# Autodesk Inventor assembly: Plate 1
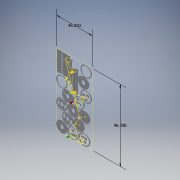
[picture p0: Inventor's stored thumbnail of the model, 180x180]
Saved by Autodesk Inventor 2016 (Build 200138000, 138)
## iProperties
Created: 2016-04-26
Part Number: Plate 1
Document SubType Name: Assembly
Designer: rubenjm
Author: rubenjm
## Documents named in this file (14)
- C:\Users\rubenjm\Documents\To Transfer\2k16 Spring\RME\GGC\V3\Plate 1.iam
- C:\Users\rubenjm\Documents\To Transfer\2k16 Spring\RME\GGC\V3\Arm Base.ipt
- C:\Users\rubenjm\Documents\To Transfer\2k16 Spring\RME\GGC\V3\Holder.ipt
- C:\Users\rubenjm\Documents\To Transfer\2k16 Spring\RME\GGC\V3\Far End Cap.ipt
- C:\Users\rubenjm\Documents\To Transfer\2k16 Spring\RME\GGC\V3\Near Holder.ipt
- C:\Users\rubenjm\Documents\To Transfer\2k16 Spring\RME\GGC\V3\Motor Bracket.ipt
- C:\Users\rubenjm\Documents\To Transfer\2k16 Spring\RME\GGC\V3\Near End Cap.ipt
- C:\Users\rubenjm\Documents\To Transfer\2k16 Spring\RME\GGC\V3\Arm Side.ipt
- C:\Users\rubenjm\Documents\To Transfer\2k16 Spring\RME\GGC\V3\Arm Top.ipt
- C:\Users\rubenjm\Documents\To Transfer\2k16 Spring\RME\GGC\V3\Turntable Top.ipt
- C:\Users\rubenjm\Documents\To Transfer\2k16 Spring\RME\GGC\V3\Turntable Sheath.ipt
- C:\Users\rubenjm\Documents\To Transfer\2k16 Spring\RME\GGC\V3\Turntable Mount.ipt
- C:\Users\rubenjm\Documents\To Transfer\2k16 Spring\RME\GGC\V3\Turntable Cap.ipt
- C:\Users\rubenjm\Documents\To Transfer\2k16 Spring\RME\GGC\V3\Turntable Mid.ipt
## Components (36 placed, 13 different names)
1. Arm Base:1 — Mate:1, Mate:59, Mate:75, Tangent:36
2. Holder:1 — Mate:4
3. Holder:2 — Mate:7
4. Far End Cap:1 — Mate:10
5. Near Holder:1 — Mate:13
6. Motor Bracket:1 — Mate:17
7. Near End Cap:1 — Mate:21
8. Arm Side:1 — Mate:25, Mate:64, Mate:69, Mate:70
9. Arm Side:2 — Mate:28, Mate:61, Mate:66, Mate:70, Mate:71
10. Arm Top:1 — Mate:30, Mate:60, Mate:72, Mate:73
11. Turntable Top:1 — Mate:33, Tangent:1, Tangent:2, Tangent:4, Tangent:10
12. Turntable Sheath:1 — Mate:34, Tangent:9, Tangent:10, Mate:41, Tangent:13, Tangent:34
13. Turntable Sheath:2 — Mate:38, Tangent:3, Tangent:4, Tangent:6, Tangent:9
14. Turntable Sheath:3 — Mate:37, Tangent:5, Tangent:6, Tangent:35
15. Turntable Sheath:4 — Mate:36, Tangent:32
16. Turntable Mount:1 — Mate:35, Mate:41
17. Turntable Cap:1 — Mate:40, Tangent:16, Tangent:19, Tangent:26
18. Turntable Mid:1 — Mate:39, Tangent:31, Tangent:32, Tangent:36
19. Arm Base:2 — Mate:55, Mate:74, Mate:75
20. Holder:3 — Mate:63
21. Holder:4 — Mate:57
22. Far End Cap:2 — Mate:53
23. Near Holder:2 — Mate:62
24. Motor Bracket:2 — Mate:52
25. Near End Cap:2 — Mate:54
26. Arm Side:3 — Mate:58, Mate:68, Mate:69
27. Arm Side:4 — Mate:65, Mate:71, Mate:72
28. Arm Top:2 — Mate:56, Mate:73, Mate:74
29. Turntable Top:2 — Tangent:13, Tangent:16, Tangent:18, Tangent:20, Mate:45, Tangent:33
30. Turntable Sheath:5 — Mate:44, Tangent:29, Tangent:30
31. Turntable Sheath:6 — Mate:43, Tangent:21, Tangent:22, Mate:50, Mate:67, Mate:76, Tangent:34
32. Turntable Sheath:7 — Mate:48, Tangent:26, Tangent:27, Tangent:28, Tangent:33
33. Turntable Sheath:8 — Mate:51, Tangent:28, Tangent:31
34. Turntable Mount:2 — Mate:46, Mate:76
35. Turntable Cap:2 — Mate:42, Tangent:19, Tangent:20, Tangent:35
36. Turntable Mid:2 — Tangent:18, Tangent:22, Mate:49, Tangent:27, Tangent:30
## Relationships (79: Mate 53, Tangent 26)
- Mate:1: Arm Base:1
- Mate:4: Holder:1
- Mate:7: Holder:2
- Mate:10: Far End Cap:1
- Mate:13: Near Holder:1
- Mate:17: Motor Bracket:1
- Mate:21: Near End Cap:1
- Mate:25: Arm Side:1
- Mate:28: Arm Side:2
- Mate:30: Arm Top:1
- Mate:33: Turntable Top:1
- Mate:34: Turntable Sheath:1
- Mate:35: Turntable Mount:1
- Mate:36: Turntable Sheath:4
- Mate:37: Turntable Sheath:3
- Mate:38: Turntable Sheath:2
- Mate:39: Turntable Mid:1
- Mate:40: Turntable Cap:1
- Tangent:1: Turntable Top:1
- Tangent:2: Turntable Top:1
- Tangent:3: Turntable Sheath:2
- Tangent:4 (6.35 mm): Turntable Top:1 ↔ Turntable Sheath:2
- Tangent:5: Turntable Sheath:3
- Tangent:6 (6.35 mm): Turntable Sheath:2 ↔ Turntable Sheath:3
- Tangent:9 (6.35 mm): Turntable Sheath:1 ↔ Turntable Sheath:2
- Tangent:10 (6.35 mm): Turntable Top:1 ↔ Turntable Sheath:1
- Mate:41: Turntable Sheath:1 ↔ Turntable Mount:1
- Tangent:13 (6.35 mm): Turntable Sheath:1 ↔ Turntable Top:2
- Tangent:16 (6.35 mm): Turntable Cap:1 ↔ Turntable Top:2
- Tangent:18 (6.35 mm): Turntable Top:2 ↔ Turntable Mid:2
- Mate:42: Turntable Cap:2
- Tangent:19 (6.35 mm): Turntable Cap:1 ↔ Turntable Cap:2
- Tangent:20 (6.35 mm): Turntable Top:2 ↔ Turntable Cap:2
- Mate:43: Turntable Sheath:6
- Tangent:21: Turntable Sheath:6
- Tangent:22 (6.35 mm): Turntable Sheath:6 ↔ Turntable Mid:2
- Mate:44: Turntable Sheath:5
- Mate:45: Turntable Top:2
- Mate:46: Turntable Mount:2
- Mate:48: Turntable Sheath:7
- Mate:49: Turntable Mid:2
- Tangent:26 (6.35 mm): Turntable Cap:1 ↔ Turntable Sheath:7
- Tangent:27 (6.35 mm): Turntable Sheath:7 ↔ Turntable Mid:2
- Mate:50: Turntable Sheath:6
- Mate:51: Turntable Sheath:8
- Tangent:28 (6.35 mm): Turntable Sheath:7 ↔ Turntable Sheath:8
- Mate:52: Motor Bracket:2
- Mate:53: Far End Cap:2
- Mate:54: Near End Cap:2
- Mate:55: Arm Base:2
- Mate:56: Arm Top:2
- Mate:57: Holder:4
- Mate:58: Arm Side:3
- Mate:59: Arm Base:1
- Mate:60: Arm Top:1
- Mate:61: Arm Side:2
- Mate:62: Near Holder:2
- Mate:63: Holder:3
- Mate:64: Arm Side:1
- Mate:65: Arm Side:4
- Mate:66: Arm Side:2
- Mate:67: Turntable Sheath:6
- Tangent:29: Turntable Sheath:5
- Tangent:30 (6.35 mm): Turntable Sheath:5 ↔ Turntable Mid:2
- Tangent:31 (6.35 mm): Turntable Mid:1 ↔ Turntable Sheath:8
- Mate:68: Arm Side:3
- Mate:69 (6.35 mm): Arm Side:1 ↔ Arm Side:3
- Mate:70 (6.35 mm): Arm Side:1 ↔ Arm Side:2
- Mate:71 (6.35 mm): Arm Side:2 ↔ Arm Side:4
- Mate:72 (6.35 mm): Arm Top:1 ↔ Arm Side:4
- Mate:73 (6.35 mm): Arm Top:1 ↔ Arm Top:2
- Mate:74 (6.35 mm): Arm Base:2 ↔ Arm Top:2
- Mate:75 (6.35 mm): Arm Base:1 ↔ Arm Base:2
- Tangent:32 (6.35 mm): Turntable Sheath:4 ↔ Turntable Mid:1
- Tangent:33 (6.35 mm): Turntable Top:2 ↔ Turntable Sheath:7
- Mate:76: Turntable Sheath:6 ↔ Turntable Mount:2
- Tangent:34 (6.35 mm): Turntable Sheath:1 ↔ Turntable Sheath:6
- Tangent:35 (6.35 mm): Turntable Sheath:3 ↔ Turntable Cap:2
- Tangent:36 (6.35 mm): Arm Base:1 ↔ Turntable Mid:1
